# Autodesk Inventor assembly: pneumatic thing 1
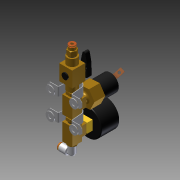
[picture p0: Inventor's stored thumbnail of the model, 180x180]
Saved by Autodesk Inventor 2014 SP1 (Build 180222100, 222)
## iProperties
Created: 2013-12-13
Part Number: pneumatic thing 1
Document SubType Name: Assembly
Designer: Moses
Mass: 1240.84 g
Surface Area: 3277.63 cm^2
Volume: 609.67 cm^3
Density: 2.03527 g/cm^3
Author: Moses
## Documents named in this file (10)
- C:\Users\Arpan\Downloads\Backup Sally 1-5-13\Backup Sally 1-5-13\pneumatic thing 1.iam
- C:\Users\Arpan\Downloads\Backup Sally 1-5-13\Backup Sally 1-5-13\Pneumatics_Parker_PV609-2.ipt
- C:\Users\Arpan\Downloads\Backup Sally 1-5-13\Backup Sally 1-5-13\Pneumatics_SMC_KQ2H03-34S.ipt
- C:\Users\Arpan\Downloads\Backup Sally 1-5-13\Backup Sally 1-5-13\Pneumatics_NASON_SM-2B-115R.ipt
- C:\Users\Arpan\Downloads\Backup Sally 1-5-13\Backup Sally 1-5-13\Pneumatics_Parker_2203P-2.ipt
- C:\Users\Arpan\Downloads\Backup Sally 1-5-13\Backup Sally 1-5-13\Pneumatics_Parker_216P-2.ipt
- C:\Users\Arpan\Downloads\Backup Sally 1-5-13\Backup Sally 1-5-13\Pneumatics_SMC_KQ2L03-34S.ipt
- C:\Users\Arpan\Downloads\Backup Sally 1-5-13\Backup Sally 1-5-13\Pneumatics_WIKA_9690242.ipt
- C:\Users\Arpan\Downloads\Backup Sally 1-5-13\Backup Sally 1-5-13\Standard #10 Washer.ipt
- C:\Users\Arpan\Downloads\Backup Sally 1-5-13\Backup Sally 1-5-13\Pneumatics Steel Bracket.ipt
## Components (15 placed, 9 different names)
1. Pneumatics_Parker_PV609-2:1 — Insert:1, Insert:3, Angle:2
2. Pneumatics_SMC_KQ2H03-34S:1 — Insert:1
3. Pneumatics_NASON_SM-2B-115R:1 — Insert:4
4. Pneumatics_Parker_2203P-2:1 — Insert:2, Insert:4, Angle:2, Insert:5, Angle:4, Tangent:6, Mate:23, Mate:24
5. Pneumatics_Parker_216P-2:1 — Insert:2, Insert:3
6. Pneumatics_Parker_216P-2:2 — Insert:5, Insert:6
7. Pneumatics_Parker_2203P-2:2 — Insert:6, Angle:4, Insert:7, Insert:8, Angle:6
8. Pneumatics_SMC_KQ2L03-34S:1 — Insert:7
9. Pneumatics_WIKA_9690242:1 — Insert:8, Angle:6
10. Pneumatics Steel Bracket:1 — Flush:4, Mate:23
11. Pneumatics Steel Bracket:2 — Tangent:6, Flush:4, Mate:24
12. Standard #10 Washer:5
13. Standard #10 Washer:6
14. Standard #10 Washer:7
15. Standard #10 Washer:8
## Relationships (15: Insert 8, Angle 3, Mate 2, Tangent 1, Flush 1)
- Insert:1 (1.27 mm): Pneumatics_Parker_PV609-2:1 ↔ Pneumatics_SMC_KQ2H03-34S:1
- Insert:2 (1.27 mm): Pneumatics_Parker_2203P-2:1 ↔ Pneumatics_Parker_216P-2:1
- Insert:3 (1.27 mm): Pneumatics_Parker_PV609-2:1 ↔ Pneumatics_Parker_216P-2:1
- Insert:4 (-1.27 mm): Pneumatics_NASON_SM-2B-115R:1 ↔ Pneumatics_Parker_2203P-2:1
- Angle:2 (0 deg): Pneumatics_Parker_PV609-2:1 ↔ Pneumatics_Parker_2203P-2:1
- Insert:5 (2.54 mm): Pneumatics_Parker_2203P-2:1 ↔ Pneumatics_Parker_216P-2:2
- Insert:6 (2.54 mm): Pneumatics_Parker_216P-2:2 ↔ Pneumatics_Parker_2203P-2:2
- Angle:4 (0 deg): Pneumatics_Parker_2203P-2:1 ↔ Pneumatics_Parker_2203P-2:2
- Insert:7 (1.27 mm): Pneumatics_Parker_2203P-2:2 ↔ Pneumatics_SMC_KQ2L03-34S:1
- Insert:8 (1.27 mm): Pneumatics_Parker_2203P-2:2 ↔ Pneumatics_WIKA_9690242:1
- Angle:6 (0 deg): Pneumatics_Parker_2203P-2:2 ↔ Pneumatics_WIKA_9690242:1
- Tangent:6: Pneumatics_Parker_2203P-2:1 ↔ Pneumatics Steel Bracket:2
- Flush:4: Pneumatics Steel Bracket:1 ↔ Pneumatics Steel Bracket:2
- Mate:23 (3.175 mm): Pneumatics_Parker_2203P-2:1 ↔ Pneumatics Steel Bracket:1
- Mate:24 (3.175 mm): Pneumatics_Parker_2203P-2:1 ↔ Pneumatics Steel Bracket:2
